# Autodesk Inventor assembly: 5-8 Rod End Assembly
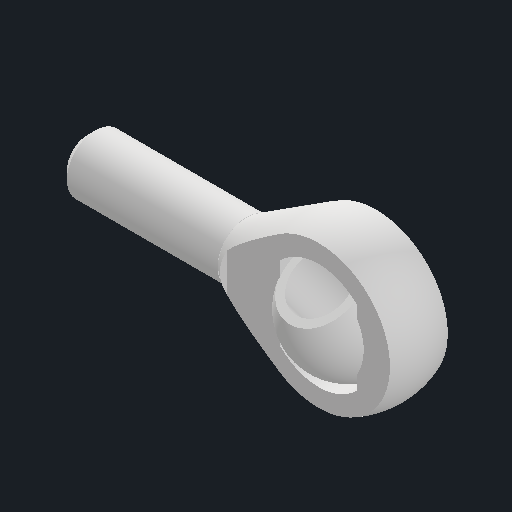
[picture p0: Inventor's stored thumbnail of the model, 512x512]
Saved by Autodesk Inventor 2026.1 (Build 301233000, 233)
## iProperties
Created: 2026-07-08
Part Number: 5-8 Rod End Assembly
Document SubType Name: Assembly
Designer: share
Author: share
## Documents named in this file (4)
- C:\Users\share\OneDrive\Documents\Personal Projects\GOGO Kart\CAD\GOGO_KART_FSAE\Rod Ends\5-8 Rod End\Suspension Rod Ends\Front Left\Upper\5-8 Rod End Assembly-Upper-FL-UOP.iam
- C:\Users\share\OneDrive\Documents\Personal Projects\GOGO Kart\CAD\GOGO_KART_FSAE\Rod Ends\5-8 Rod End\5-8 Rod End Ball Correct.ipt
- C:\Users\share\OneDrive\Documents\Personal Projects\GOGO Kart\CAD\GOGO_KART_FSAE\Rod Ends\5-8 Rod End\5-8 Rod End Head Correct.ipt
- C:\Users\share\OneDrive\Documents\Personal Projects\GOGO Kart\CAD\GOGO_KART_FSAE\Rod Ends\5-8 Rod End\5-8 Rod End Rod Correct.ipt
## Components (3 placed, 3 different names)
1. 5-8 Rod End Ball Correct:1 — Mate:3
2. 5-8 Rod End Head Correct:1 — Flush:1, Mate:1, Mate:2, Insert:1, Mate:3
3. 5-8 Rod End Rod Correct:1 — Insert:1
## Relationships (5: Mate 3, Flush 1, Insert 1)
- Flush:1: 5-8 Rod End Head Correct:1
- Mate:1: 5-8 Rod End Head Correct:1
- Mate:2: 5-8 Rod End Head Correct:1
- Insert:1: 5-8 Rod End Head Correct:1 ↔ 5-8 Rod End Rod Correct:1
- Mate:3: 5-8 Rod End Ball Correct:1 ↔ 5-8 Rod End Head Correct:1
